# Autodesk Inventor assembly: macropad
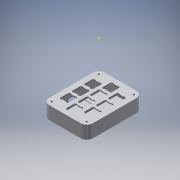
[picture p0: Inventor's stored thumbnail of the model, 180x180]
Saved by Autodesk Inventor 2019 (Build 230136000, 136)
## iProperties
Created: 2019-01-13
Part Number: macropad
Document SubType Name: Assembly
Designer: onemo
Author: onemo
## Documents named in this file (3)
- D:\Code\school\ieee\Macropad\case\cad\macropad.iam
- D:\Code\school\ieee\Macropad\case\cad\macropad-frame.ipt
- D:\Code\school\ieee\Macropad\case\cad\macropad-plate-01.ipt
## Components (2 placed, 2 different names)
1. macropad-frame:1 — Flush:1, Flush:2, Mate:1
2. macropad-plate-01:1 — Flush:1, Flush:2, Mate:1
## Relationships (3: Flush 2, Mate 1)
- Flush:1: macropad-frame:1 ↔ macropad-plate-01:1
- Flush:2: macropad-frame:1 ↔ macropad-plate-01:1
- Mate:1: macropad-frame:1 ↔ macropad-plate-01:1
